# Autodesk Inventor assembly: hotend_assembly
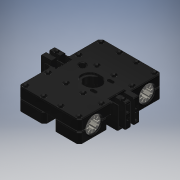
[picture p0: Inventor's stored thumbnail of the model, 180x180]
Saved by Autodesk Inventor 2018 (Build 220112000, 112)
## iProperties
Created: 2018-07-15
Part Number: hotend_assembly
Document SubType Name: Assembly
Designer: Z. Deniz
Author: Z. Deniz
## Documents named in this file (6)
- C:\Users\zdeni\Desktop\3d\Yeni klasör\hotend_assembly.iam
- C:\Users\zdeni\Desktop\3d\Yeni klasör\hotend_holder.ipt
- C:\Users\zdeni\Desktop\3d\Yeni klasör\hotend_holder_clamp.ipt
- C:\Users\zdeni\Desktop\3d\Yeni klasör\123RJ4JP_01_08_1.ipt
- C:\Users\zdeni\Desktop\3d\Yeni klasör\hotend_holder_pulley.ipt
- C:\Users\zdeni\Desktop\3d\Yeni klasör\hotend__belt_holder.ipt
## Components (14 placed, 5 different names)
1. hotend_holder:1 — Mate:2, Mate:3, Mate:5, Mate:7, Mate:9, Mate:10, Mate:11, Mate:12, Mate:13, Flush:1, Flush:2, Flush:3, Flush:4, Flush:5, Flush:6, Flush:7, Flush:8, Mate:18, Mate:19, Mate:20, Mate:24, Mate:25, Mate:28, Mate:29, Mate:30, Mate:31, Mate:32, Mate:33, Mate:34, Mate:35
2. hotend_holder_clamp:1 — Mate:2, Mate:35
3. 123RJ4JP_01_08_1:1 — Mate:5, Mate:10, Mate:15
4. 123RJ4JP_01_08_1:2 — Mate:3, Mate:11, Mate:14
5. 123RJ4JP_01_08_1:3 — Mate:7, Mate:12, Mate:17
6. 123RJ4JP_01_08_1:4 — Mate:9, Mate:13, Mate:16
7. hotend_holder_pulley:1 — Mate:15, Flush:2, Flush:8
8. hotend_holder_pulley:2 — Mate:17, Flush:4, Flush:5
9. hotend_holder_pulley:3 — Mate:16, Flush:3, Flush:6
10. hotend_holder_pulley:4 — Mate:14, Flush:1, Flush:7
11. hotend__belt_holder:1 — Mate:24, Mate:25, Mate:28
12. hotend__belt_holder:2 — Mate:18, Mate:19, Mate:20
13. hotend__belt_holder:3 — Mate:29, Mate:30, Mate:31
14. hotend__belt_holder:4 — Mate:32, Mate:33, Mate:34
## Relationships (34: Mate 26, Flush 8)
- Mate:2 (0.25 mm): hotend_holder:1 ↔ hotend_holder_clamp:1
- Mate:3: hotend_holder:1 ↔ 123RJ4JP_01_08_1:2
- Mate:5: hotend_holder:1 ↔ 123RJ4JP_01_08_1:1
- Mate:7: hotend_holder:1 ↔ 123RJ4JP_01_08_1:3
- Mate:9: hotend_holder:1 ↔ 123RJ4JP_01_08_1:4
- Mate:10: hotend_holder:1 ↔ 123RJ4JP_01_08_1:1
- Mate:11: hotend_holder:1 ↔ 123RJ4JP_01_08_1:2
- Mate:12: hotend_holder:1 ↔ 123RJ4JP_01_08_1:3
- Mate:13: hotend_holder:1 ↔ 123RJ4JP_01_08_1:4
- Mate:14: 123RJ4JP_01_08_1:2 ↔ hotend_holder_pulley:4
- Flush:1: hotend_holder:1 ↔ hotend_holder_pulley:4
- Mate:15: 123RJ4JP_01_08_1:1 ↔ hotend_holder_pulley:1
- Mate:16: 123RJ4JP_01_08_1:4 ↔ hotend_holder_pulley:3
- Mate:17: 123RJ4JP_01_08_1:3 ↔ hotend_holder_pulley:2
- Flush:2: hotend_holder:1 ↔ hotend_holder_pulley:1
- Flush:3: hotend_holder:1 ↔ hotend_holder_pulley:3
- Flush:4: hotend_holder:1 ↔ hotend_holder_pulley:2
- Flush:5: hotend_holder:1 ↔ hotend_holder_pulley:2
- Flush:6: hotend_holder:1 ↔ hotend_holder_pulley:3
- Flush:7: hotend_holder:1 ↔ hotend_holder_pulley:4
- Flush:8: hotend_holder:1 ↔ hotend_holder_pulley:1
- Mate:18: hotend_holder:1 ↔ hotend__belt_holder:2
- Mate:19 (5 mm): hotend_holder:1 ↔ hotend__belt_holder:2
- Mate:20 (0.25 mm): hotend_holder:1 ↔ hotend__belt_holder:2
- Mate:24 (0.25 mm): hotend_holder:1 ↔ hotend__belt_holder:1
- Mate:25 (5 mm): hotend_holder:1 ↔ hotend__belt_holder:1
- Mate:28: hotend_holder:1 ↔ hotend__belt_holder:1
- Mate:29: hotend_holder:1 ↔ hotend__belt_holder:3
- Mate:30 (0.25 mm): hotend_holder:1 ↔ hotend__belt_holder:3
- Mate:31 (5 mm): hotend_holder:1 ↔ hotend__belt_holder:3
- Mate:32: hotend_holder:1 ↔ hotend__belt_holder:4
- Mate:33 (0.25 mm): hotend_holder:1 ↔ hotend__belt_holder:4
- Mate:34 (5 mm): hotend_holder:1 ↔ hotend__belt_holder:4
- Mate:35: hotend_holder:1 ↔ hotend_holder_clamp:1
